# Autodesk Inventor assembly: ASY TZS FDS way1
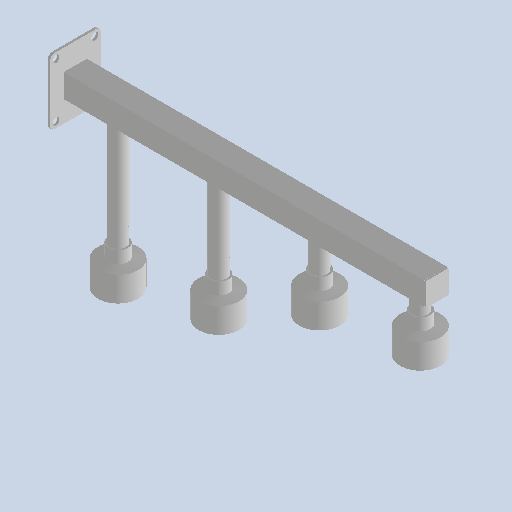
[picture p0: Inventor's stored thumbnail of the model, 512x512]
Saved by Autodesk Inventor 2025 (Build 290162010, 162A)
## iProperties
Created: 2025-07-02
Part Number: ASY TZS FDS way1
Document SubType Name: Assembly
Designer: user
Author: user
## Documents named in this file (9)
- C:\Users\pokla\Documents\Inventor\TZS-Tazovskiy\Filter D940\FDS 940\ASY TZS FDS way1.iam
- C:\Users\pokla\Documents\Inventor\TZS-Tazovskiy\Filter D940\FDS 940\TZS 754 FDS 940 way tube 1.ipt
- C:\Users\pokla\Documents\Inventor\TZS-Tazovskiy\Filter D940\FDS 940\TZS dummy filter element.ipt
- C:\Users\pokla\Documents\Inventor\TZS-Tazovskiy\Filter D940\FDS 940\TZS dummy pipe nippel.ipt
- C:\Users\pokla\Documents\Inventor\TZS-Tazovskiy\Filter D940\FDS 940\TZS 757 FDS 940 way tube 4.ipt
- C:\Users\pokla\Documents\Inventor\TZS-Tazovskiy\Filter D940\FDS 940\TZS 1756 FDS 940 way tube 6.ipt
- C:\Users\pokla\Documents\Inventor\TZS-Tazovskiy\Filter D940\FDS 940\TZS 1757 FDS 940 way tube 7.ipt
- C:\Users\pokla\Documents\Inventor\TZS-Tazovskiy\Filter D940\FDS 940\TZS 760 FDS 940 FLANGE 3.ipt
- C:\Users\pokla\Documents\Inventor\TZS-Tazovskiy\Filter D940\FDS 940\TZS 766 FDS 940 CUP 1.ipt
## Components (14 placed, 8 different names)
1. TZS 754 FDS 1200 way tube 1.ipt:1 — Rigid:13
2. TZS dummy filter element.ipt:1
3. TZS dummy pipe nippel.ipt:1
4. TZS 757 FDS 1200 way tube 4.ipt:1
5. TZS dummy filter element.ipt:2
6. TZS dummy pipe nippel.ipt:2
7. TZS 1756 FDS 1200 way tube 6.ipt:1
8. TZS dummy filter element.ipt:3
9. TZS dummy pipe nippel.ipt:3
10. TZS 1757 FDS 1200 way tube 7.ipt:1
11. TZS dummy filter element.ipt:4
12. TZS dummy pipe nippel.ipt:4
13. TZS 760 FDS 1200 FLANGE 3.ipt:1
14. TZS 766 FDS 1200 CUP 1.ipt:1 — Rigid:13
## Relationships (13: WeldJoint 13)
- [WeldJoint]: TZS dummy filter element.ipt:1 ↔ TZS dummy pipe nippel.ipt:1
- [WeldJoint]: TZS 754 FDS 1200 way tube 1.ipt:1 ↔ TZS dummy pipe nippel.ipt:1
- [WeldJoint]: TZS dummy filter element.ipt:2 ↔ TZS dummy pipe nippel.ipt:2
- [WeldJoint]: TZS 757 FDS 1200 way tube 4.ipt:1 ↔ TZS dummy pipe nippel.ipt:2
- [WeldJoint]: TZS 754 FDS 1200 way tube 1.ipt:1 ↔ TZS 757 FDS 1200 way tube 4.ipt:1
- [WeldJoint]: TZS dummy filter element.ipt:3 ↔ TZS dummy pipe nippel.ipt:3
- [WeldJoint]: TZS 1756 FDS 1200 way tube 6.ipt:1 ↔ TZS dummy pipe nippel.ipt:3
- [WeldJoint]: TZS dummy filter element.ipt:4 ↔ TZS dummy pipe nippel.ipt:4
- [WeldJoint]: TZS 1757 FDS 1200 way tube 7.ipt:1 ↔ TZS dummy pipe nippel.ipt:4
- [WeldJoint]: TZS 754 FDS 1200 way tube 1.ipt:1 ↔ TZS 1756 FDS 1200 way tube 6.ipt:1
- [WeldJoint]: TZS 754 FDS 1200 way tube 1.ipt:1 ↔ TZS 1757 FDS 1200 way tube 7.ipt:1
- [WeldJoint] (-2 mm): TZS 754 FDS 1200 way tube 1.ipt:1 ↔ TZS 760 FDS 1200 FLANGE 3.ipt:1
- Rigid:13 [WeldJoint]: TZS 754 FDS 1200 way tube 1.ipt:1 ↔ TZS 766 FDS 1200 CUP 1.ipt:1
## Named parameters: d33_d31 = 0 mm, d37_d34_d31 = 0 mm, d43_d40_d37_d34_d31 = 0 mm, d44_d41 = 0 mm, d47_d45_d43_d40_d37_d34_d31 = 0 mm, d48_d46 = 0 mm
